# Autodesk Inventor assembly: Kroller1
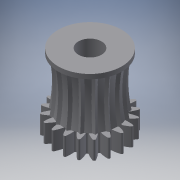
[picture p0: Inventor's stored thumbnail of the model, 180x180]
Saved by Autodesk Inventor 2016 (Build 200138000, 138)
## iProperties
Created: 2018-02-08
Part Number: Kroller1
Document SubType Name: Assembly
Designer: Simon
Author: Simon
## Documents named in this file (3)
- D:\Cad\Gymnasieprojekt\Kroller1.iam
- D:\Cad\Gymnasieprojekt\Kugg.ipt
- D:\Cad\Gymnasieprojekt\Roller_v3.ipt
## Components (2 placed, 2 different names)
1. Kugg:1 — Insert:1, Flush:1
2. Roller_v3:1 — Insert:1, Flush:1
## Relationships (2: Insert 1, Flush 1)
- Insert:1: Kugg:1 ↔ Roller_v3:1
- Flush:1: Kugg:1 ↔ Roller_v3:1
